# Autodesk Inventor assembly: Handle_ASAP2
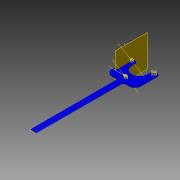
[picture p0: Inventor's stored thumbnail of the model, 180x180]
Saved by Autodesk Inventor 2011 SP2 (Build 150309200, 309)
## iProperties
Created: 2013-03-01
Part Number: Handle_ASAP2
Document SubType Name: Assembly
Designer: sungwook
Author: sungwook
## Documents named in this file (4)
- C:\Users\sungwook\Documents\Inventor\Micron22_top_adj_02082013\Parts\ASAP\Handle_ASAP2.iam
- C:\Users\sungwook\Documents\Inventor\Micron22_top_adj_02082013\Parts\ASAP\ASAP_Handle_Fixture_New2_1.ipt
- C:\Users\sungwook\Documents\Inventor\Micron22_top_adj_02082013\Parts\ASAP\LED2.ipt
- C:\Users\sungwook\Documents\Inventor\Micron22_top_adj_02082013\Parts\ASAP\LED2_MIR2.ipt
## Components (4 placed, 3 different names)
1. ASAP_Handle_Fixture_New2_1:1 — Flush:1, Mate:3, Flush:3, Mate:5, Mate:7, Flush:8
2. LED2:1 — Mate:2, Mate:3, Flush:4
3. LED2:2 — Mate:5, Mate:6, Flush:8
4. LED2_MIR2:1 — Flush:2, Mate:7, Flush:4
## Relationships (10: Flush 5, Mate 5)
- Flush:1 (-2.25 mm): ASAP_Handle_Fixture_New2_1:1
- Mate:2: LED2:1
- Mate:3: ASAP_Handle_Fixture_New2_1:1 ↔ LED2:1
- Flush:2: LED2_MIR2:1
- Flush:3 (-4 mm): ASAP_Handle_Fixture_New2_1:1
- Mate:5: ASAP_Handle_Fixture_New2_1:1 ↔ LED2:2
- Mate:6: LED2:2
- Mate:7: ASAP_Handle_Fixture_New2_1:1 ↔ LED2_MIR2:1
- Flush:4: LED2:1 ↔ LED2_MIR2:1
- Flush:8 (-13.5 mm): ASAP_Handle_Fixture_New2_1:1 ↔ LED2:2
